# Autodesk Inventor assembly: PQ60 EPS FV4.brd
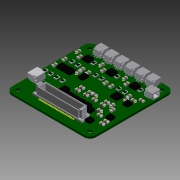
[picture p0: Inventor's stored thumbnail of the model, 180x180]
Saved by Autodesk Inventor 2015 SP1 (Build 190203100, 203)
## iProperties
Created: 2015-10-19
Part Number: PQ60 EPS FV4.brd
Document SubType Name: Assembly
Designer: Kartikye
Author: Kartikye
## Documents named in this file (17)
- C:\Users\Kartikye\Documents\GitHub\SASSat\Structure\EPS\PQ60 EPS FV4.brd.iam
- C:\Users\Kartikye\Documents\GitHub\SASSat\Structure\EPS\Parts\PQ60 EPS FV4.brd_Outline.ipt
- C:\Users\Kartikye\Documents\GitHub\SASSat\Structure\EPS\Parts\IND_ELL6XH, 10UH_40.ipt
- C:\Users\Kartikye\Documents\GitHub\SASSat\Structure\EPS\Parts\IND_ELL3FU, 2_2UH_44.ipt
- C:\Users\Kartikye\Documents\GitHub\SASSat\Structure\EPS\Parts\SOT95P237X112-3N, MCP130T-315I_TT_86.ipt
- C:\Users\Kartikye\Documents\GitHub\SASSat\Structure\EPS\Parts\DFN300X300X80-11N, LTC3105EDDPBF_102.ipt
- C:\Users\Kartikye\Documents\GitHub\SASSat\Structure\EPS\Parts\DFN300X300X80-11N, LTC4413EDDPBF_106.ipt
- C:\Users\Kartikye\Documents\GitHub\SASSat\Structure\EPS\Parts\SON50P300X300X100-11N, TPS63001DRCR_109.ipt
- C:\Users\Kartikye\Documents\GitHub\SASSat\Structure\EPS\Parts\DRV, DRV_111.ipt
- C:\Users\Kartikye\Documents\GitHub\SASSat\Structure\EPS\Parts\SON50P200X300X80-11N, BQ24210DQCT_114.ipt
- C:\Users\Kartikye\Documents\GitHub\SASSat\Structure\EPS\Parts\SOP65P640X110-16N, PCA9534PW_116.ipt
- C:\Users\Kartikye\Documents\GitHub\SASSat\Structure\Imported Components\RES0805\RES0805.ipt
- C:\Users\Kartikye\Documents\GitHub\SASSat\Structure\Imported Components\FX8C-60S-SV\FX8C-60S-SV.iam
- C:\Users\Kartikye\Documents\GitHub\SASSat\Structure\Imported Components\FX8C-60P-SV\FX8C-60P-SV.iam
- C:\Users\Kartikye\Documents\GitHub\SASSat\Structure\Imported Components\0805_cap_T0.85\0805_cap_T0.85.ipt
- C:\Users\Kartikye\Documents\GitHub\SASSat\Structure\Imported Components\SM02B-SRSS-TB\SM02B-SRSS-TB.ipt
- C:\Users\Kartikye\Documents\GitHub\SASSat\Structure\Imported Components\SM03B-SRSS-TB\SM03B-SRSS-TB.ipt
## Components (102 placed, 102 different names)
1. PQ60 EPS FV4.brd_Outline:1 — Insert:1, Insert:2, Mate:1, Insert:3, Insert:4, Mate:2, Mate:3, Mate:4, Mate:5, Mate:6, Mate:7, Flush:7, Mate:13, Flush:8, Flush:9, Mate:14, Flush:10
2. C1_2
3. C2_3
4. C3_4
5. C4_5
6. C5_6
7. C6_7
8. C7_9
9. C8_10
10. C9_11
11. C10_12
12. C11_13
13. C12_14
14. C13_15
15. C14_17
16. C15_18
17. C16_19
18. C17_20
19. C18_22
20. C19_23
21. C20_24
22. C21_25
23. C22_26
24. C23_27
25. C24_28
26. C25_29
27. C26_30
28. C27_31
29. C28_32
30. C29_33
31. C30_34
32. C31_35
33. C32_36
34. C33_37
35. C34_38
36. C35_39
37. L1_41
38. L2_42
39. L3_43
40. L4_45
41. R1_47
42. R2_48
43. R3_50
44. R4_52
45. R5_53
46. R6_54
47. R7_55
48. R8_56
49. R9_58
50. R10_60
51. R11_61
52. R12_62
53. R13_63
54. R14_64
55. R15_66
56. R16_67
57. R17_68
58. R18_70
59. R19_72
60. R20_73
61. R21_74
62. R22_75
63. R23_76
64. R24_77
65. R25_78
66. R26_79
67. R27_80
68. R28_81
69. R30_82
70. R31_83
71. R32_84
72. R33_85
73. U_1_87
74. U_4_93 — Mate:2, Flush:2, Mate:8
75. U_5_94 — Mate:3, Flush:2, Flush:3, Mate:8, Mate:9
76. U_6_95 — Mate:5, Flush:4, Flush:5, Mate:10, Mate:11
77. U_7_96 — Mate:4, Flush:3, Flush:4, Mate:9, Mate:10
78. U_8_97 — Mate:6, Flush:5, Flush:6, Mate:11, Mate:12
79. U_9_98 — Mate:7, Flush:6, Mate:12
80. U_10_99 — Flush:7, Mate:13, Flush:8
81. U_11_101 — Flush:9, Mate:14, Flush:10
82. U1_103
83. U2_104
84. U3_105
85. U4_107
86. U5_108
87. U6_110
88. U7_112
89. U8_113
90. U9_115
91. U10_117
92. U11_118
93. U12_119
94. U13_120
95. U14_121
96. U15_122
97. U16_123
98. U17_124
99. U18_125
100. U19_126
101. FX8C-60S-SV:1 [sub-assembly] — Insert:1, Insert:2
102. FX8C-60P-SV:1 [sub-assembly] — Mate:1, Insert:3, Insert:4
## Relationships (28: Mate 14, Flush 10, Insert 4)
- Insert:1: PQ60 EPS FV4.brd_Outline:1 ↔ FX8C-60S-SV:1
- Insert:2: PQ60 EPS FV4.brd_Outline:1 ↔ FX8C-60S-SV:1
- Mate:1: PQ60 EPS FV4.brd_Outline:1 ↔ FX8C-60P-SV:1
- Insert:3: PQ60 EPS FV4.brd_Outline:1 ↔ FX8C-60P-SV:1
- Insert:4: PQ60 EPS FV4.brd_Outline:1 ↔ FX8C-60P-SV:1
- Mate:2: PQ60 EPS FV4.brd_Outline:1 ↔ U_4_93
- [Flush]: U_4_93 ↔ U_5_94
- Mate:3: PQ60 EPS FV4.brd_Outline:1 ↔ U_5_94
- Flush:2: U_4_93 ↔ U_5_94
- Mate:4: PQ60 EPS FV4.brd_Outline:1 ↔ U_7_96
- Mate:5: PQ60 EPS FV4.brd_Outline:1 ↔ U_6_95
- Flush:3: U_5_94 ↔ U_7_96
- Mate:6: PQ60 EPS FV4.brd_Outline:1 ↔ U_8_97
- Flush:4: U_6_95 ↔ U_7_96
- Flush:5: U_6_95 ↔ U_8_97
- Mate:7: PQ60 EPS FV4.brd_Outline:1 ↔ U_9_98
- Flush:6: U_8_97 ↔ U_9_98
- Mate:8 (1.2 mm): U_4_93 ↔ U_5_94
- Mate:9 (1.2 mm): U_5_94 ↔ U_7_96
- Mate:10 (1.2 mm): U_6_95 ↔ U_7_96
- Mate:11 (1.2 mm): U_6_95 ↔ U_8_97
- Mate:12 (1.2 mm): U_8_97 ↔ U_9_98
- Flush:7 (6.05 mm): PQ60 EPS FV4.brd_Outline:1 ↔ U_10_99
- Mate:13: PQ60 EPS FV4.brd_Outline:1 ↔ U_10_99
- Flush:8 (0.7 mm): PQ60 EPS FV4.brd_Outline:1 ↔ U_10_99
- Flush:9 (9.95 mm): PQ60 EPS FV4.brd_Outline:1 ↔ U_11_101
- Mate:14: PQ60 EPS FV4.brd_Outline:1 ↔ U_11_101
- Flush:10 (0.7 mm): PQ60 EPS FV4.brd_Outline:1 ↔ U_11_101
